# Autodesk Inventor assembly: main
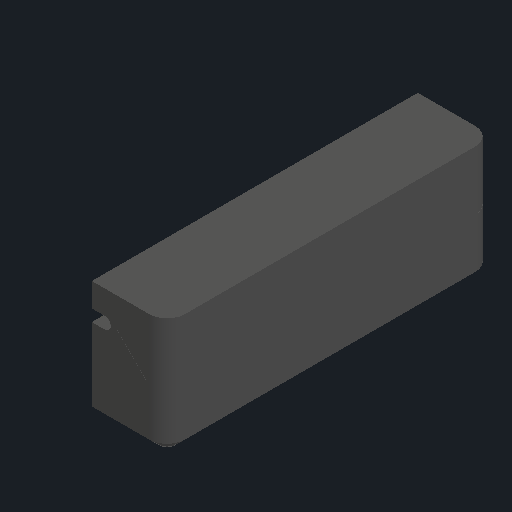
[picture p0: Inventor's stored thumbnail of the model, 512x512]
Saved by Autodesk Inventor 2026.2 (Build 302298000, 298)
## iProperties
Created: 2025-12-22
Part Number: main
Document SubType Name: Assembly
Designer: test
Author: test
## Documents named in this file (6)
- D:\Projects\WearableWLED\WearableWLED_Mechanical\main.iam
- D:\Projects\WearableWLED\WearableWLED_Mechanical\case1.ipt
- D:\Projects\WearableWLED\WearableWLED_Mechanical\battery.ipt
- D:\Projects\WearableWLED\WearableWLED_Mechanical\case2.ipt
- D:\Projects\WearableWLED\WearableWLED_Mechanical\board\WearableWLED_Hardware\WearableWLED_Hardware\WearableWLED_Hardware.iam
- D:\Projects\WearableWLED\WearableWLED_Mechanical\dimmensions.xlsx
## Components (4 placed, 4 different names)
1. case1:1 — Mate:2, Mate:3, Mate:4, Flush:1, Flush:2, Mate:8
2. battery:1 — Mate:2, Mate:3, Mate:4
3. case2:1 — Mate:5, Mate:6, Mate:7, Flush:1, Flush:2, Mate:8
4. WearableWLED_Hardware:1 [sub-assembly] — Mate:5, Mate:6, Mate:7
## Relationships (9: Mate 7, Flush 2)
- Mate:2: case1:1 ↔ battery:1
- Mate:3 (0.5 mm): case1:1 ↔ battery:1
- Mate:4 (0.5 mm): case1:1 ↔ battery:1
- Mate:5 (0.5 mm): case2:1 ↔ WearableWLED_Hardware:1
- Mate:6: case2:1 ↔ WearableWLED_Hardware:1
- Mate:7: case2:1 ↔ WearableWLED_Hardware:1
- Flush:1: case1:1 ↔ case2:1
- Flush:2: case1:1 ↔ case2:1
- Mate:8: case1:1 ↔ case2:1
## Named parameters: wall_thickness = 2 mm, case_h = 16 mm, case_d = 51 mm, case_w = 21 mm, case_ratio = 0.5, case_mounting = 0.8 mm
note: some values were not read from the file. Shown as the stored number, unit unknown: "case_ratio".
